# Autodesk Inventor assembly: Chasis inferior _1_
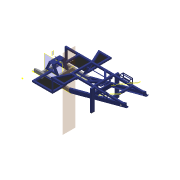
[picture p0: Inventor's stored thumbnail of the model, 180x180]
Saved by Autodesk Inventor 2020 (Build 240168000, 168)
## iProperties
Created: 2020-02-06
Part Number: Chasis inferior _1_
Document SubType Name: Assembly
Designer: Juan Carlos Botero
Author: Juan Carlos Botero
## Documents named in this file (46)
- D:\Drives\OneDrive\Carlos_2\02 TRABAJOS\MULTIPLO\Conveyor\ENSAMBLE\Chasis inferior _1_.iam
- D:\Drives\OneDrive\Carlos_2\02 TRABAJOS\MULTIPLO\Conveyor\ENSAMBLE\Refuerzo diagonal tiro.ipt
- D:\Drives\OneDrive\Carlos_2\02 TRABAJOS\MULTIPLO\Conveyor\ENSAMBLE\Lamina escalon 2.ipt
- D:\Drives\OneDrive\Carlos_2\02 TRABAJOS\MULTIPLO\Conveyor\ENSAMBLE\Lamina sujeción bateria 2.ipt
- D:\Drives\OneDrive\Carlos_2\02 TRABAJOS\MULTIPLO\Conveyor\ENSAMBLE\Refuerzo perfil en C.ipt
- D:\Drives\OneDrive\Carlos_2\02 TRABAJOS\MULTIPLO\Conveyor\ENSAMBLE\Tapa perfil 100x50.ipt
- D:\Drives\OneDrive\Carlos_2\02 TRABAJOS\MULTIPLO\Conveyor\ENSAMBLE\Angulo soporte batería 1.ipt
- D:\Drives\OneDrive\Carlos_2\02 TRABAJOS\MULTIPLO\Conveyor\ENSAMBLE\Perfil 1 en C derecho 2.ipt
- D:\Drives\OneDrive\Carlos_2\02 TRABAJOS\MULTIPLO\Conveyor\ENSAMBLE\Caucho tope banda.ipt
- D:\Drives\OneDrive\Carlos_2\02 TRABAJOS\MULTIPLO\Conveyor\ENSAMBLE\Refuerzo diagonal chasis inferior.ipt
- D:\Drives\OneDrive\Carlos_2\02 TRABAJOS\MULTIPLO\Conveyor\ENSAMBLE\Perfil escalón 6.ipt
- D:\Drives\OneDrive\Carlos_2\02 TRABAJOS\MULTIPLO\Conveyor\ENSAMBLE\Perfil escalón 3.ipt
- D:\Drives\OneDrive\Carlos_2\02 TRABAJOS\MULTIPLO\Conveyor\ENSAMBLE\Espaciador de nylon.ipt
- D:\Drives\OneDrive\Carlos_2\02 TRABAJOS\MULTIPLO\Conveyor\ENSAMBLE\Refuerzo chasis.ipt
- D:\Drives\OneDrive\Carlos_2\02 TRABAJOS\MULTIPLO\Conveyor\ENSAMBLE\Perfil escalón 4.ipt
- D:\Drives\OneDrive\Carlos_2\02 TRABAJOS\MULTIPLO\Conveyor\ENSAMBLE\Tope banda.ipt
- D:\Drives\OneDrive\Carlos_2\02 TRABAJOS\MULTIPLO\Conveyor\ENSAMBLE\Buje.ipt
- D:\Drives\OneDrive\Carlos_2\02 TRABAJOS\MULTIPLO\Conveyor\ENSAMBLE\Lamina indexacion eje trasero.ipt
- D:\Drives\OneDrive\Carlos_2\02 TRABAJOS\MULTIPLO\Conveyor\ENSAMBLE\Refuerzo horizontal tiro.ipt
- D:\Drives\OneDrive\Carlos_2\02 TRABAJOS\MULTIPLO\Conveyor\ENSAMBLE\Angulo escalón 1.ipt
- D:\Drives\OneDrive\Carlos_2\02 TRABAJOS\MULTIPLO\Conveyor\ENSAMBLE\Base chasis inferior izquierdo.ipt
- D:\Drives\OneDrive\Carlos_2\02 TRABAJOS\MULTIPLO\Conveyor\ENSAMBLE\Refuerzo diagonal estructura tiro.ipt
- D:\Drives\OneDrive\Carlos_2\02 TRABAJOS\MULTIPLO\Conveyor\ENSAMBLE\Perfil 1 en C izquierdo 2.ipt
- D:\Drives\OneDrive\Carlos_2\02 TRABAJOS\MULTIPLO\Conveyor\ENSAMBLE\Lamina escalon 1.ipt
- D:\Drives\OneDrive\Carlos_2\02 TRABAJOS\MULTIPLO\Conveyor\ENSAMBLE\Lamina pivote actuador lineal pequeño.ipt
- D:\Drives\OneDrive\Carlos_2\02 TRABAJOS\MULTIPLO\Conveyor\ENSAMBLE\Perfil 1 en C izquierdo 1.ipt
- D:\Drives\OneDrive\Carlos_2\02 TRABAJOS\MULTIPLO\Conveyor\ENSAMBLE\Perfil 1 en C derecho 1.ipt
- D:\Drives\OneDrive\Carlos_2\02 TRABAJOS\MULTIPLO\Conveyor\ENSAMBLE\Perfil escalón 2.ipt
- D:\Drives\OneDrive\Carlos_2\02 TRABAJOS\MULTIPLO\Conveyor\ENSAMBLE\Espaciador pivote 1.ipt
- D:\Drives\OneDrive\Carlos_2\02 TRABAJOS\MULTIPLO\Conveyor\ENSAMBLE\Platina inferior actuador lineal.ipt
- D:\Drives\OneDrive\Carlos_2\02 TRABAJOS\MULTIPLO\Conveyor\ENSAMBLE\Angulo escalón 3.ipt
- D:\Drives\OneDrive\Carlos_2\02 TRABAJOS\MULTIPLO\Conveyor\ENSAMBLE\Refuerzo diagonal.ipt
- D:\Drives\OneDrive\Carlos_2\02 TRABAJOS\MULTIPLO\Conveyor\ENSAMBLE\Perfil escalón 1.ipt
- D:\Drives\OneDrive\Carlos_2\02 TRABAJOS\MULTIPLO\Conveyor\ENSAMBLE\Pie amigo lamina quinta rueda.ipt
- D:\Drives\OneDrive\Carlos_2\02 TRABAJOS\MULTIPLO\Conveyor\ENSAMBLE\Lamina pivote quinta rueda.ipt
- D:\Drives\OneDrive\Carlos_2\02 TRABAJOS\MULTIPLO\Conveyor\ENSAMBLE\Angulo soporte batería 3.ipt
- D:\Drives\OneDrive\Carlos_2\02 TRABAJOS\MULTIPLO\Conveyor\ENSAMBLE\Angulo soporte batería 2.ipt
- D:\Drives\OneDrive\Carlos_2\02 TRABAJOS\MULTIPLO\Conveyor\ENSAMBLE\Unión base chasis inferior.ipt
- D:\Drives\OneDrive\Carlos_2\02 TRABAJOS\MULTIPLO\Conveyor\ENSAMBLE\Base chasis inferior derecho.ipt
- D:\Drives\OneDrive\Carlos_2\02 TRABAJOS\MULTIPLO\Conveyor\ENSAMBLE\Refuerzo intermedio.ipt
- D:\Drives\OneDrive\Carlos_2\02 TRABAJOS\MULTIPLO\Conveyor\ENSAMBLE\Ensamble cuñas y soporte _1_.iam
- D:\Drives\OneDrive\Carlos_2\02 TRABAJOS\MULTIPLO\Conveyor\ENSAMBLE\Ensamble cuñas y soporte _1__1.iam
- D:\Drives\OneDrive\Carlos_2\02 TRABAJOS\MULTIPLO\Conveyor\ENSAMBLE\sketch.ipt
- D:\Drives\OneDrive\Carlos_2\02 TRABAJOS\MULTIPLO\Conveyor\ENSAMBLE\Perfil 1 en C derecho 2_MIR.ipt
- D:\Drives\OneDrive\Carlos_2\02 TRABAJOS\MULTIPLO\Paral_baliza.iam
- D:\Drives\OneDrive\Carlos_2\02 TRABAJOS\MULTIPLO\Conveyor\ENSAMBLE - Copy\Modificacion_altura.iam
## Components (80 placed, 44 different names)
1. Refuerzo diagonal tiro:1
2. Lamina escalon 2:1
3. Lamina sujeción bateria 2:1
4. Lamina escalon 2:2
5. Refuerzo perfil en C:1
6. Tapa perfil 100x50:1
7. Angulo soporte batería 1:1
8. Perfil 1 en C derecho 2:1
9. Caucho tope banda:1
10. Refuerzo diagonal chasis inferior:1
11. Perfil escalón 6:1
12. Refuerzo perfil en C:2
13. Espaciador de nylon:1
14. Perfil escalón 4:1
15. Tope banda:1
16. Buje:1
17. Perfil escalón 3:2
18. Lamina indexacion eje trasero:1
19. Refuerzo horizontal tiro:1
20. Angulo escalón 1:1
21. Base chasis inferior izquierdo:1
22. Perfil escalón 3:3
23. Lamina indexacion eje trasero:2
24. Refuerzo horizontal tiro:2 — Flush:7
25. Caucho tope banda:2
26. Refuerzo diagonal estructura tiro:1
27. Refuerzo diagonal tiro:2
28. Perfil 1 en C izquierdo 2:1
29. Tapa perfil 100x50:2
30. Refuerzo diagonal chasis inferior:2
31. Lamina escalon 1:1
32. Lamina pivote actuador lineal pequeño:1
33. Perfil 1 en C izquierdo 1:1
34. Perfil 1 en C derecho 1:1
35. Perfil escalón 2:1 — Flush:14, Flush:15
36. Lamina pivote actuador lineal pequeño:2
37. Espaciador pivote 1:1
38. Refuerzo chasis:2
39. Perfil escalón 3:4
40. Platina inferior actuador lineal:1
41. Espaciador pivote 1:2
42. Buje:3
43. Perfil escalón 3:5
44. Angulo escalón 3:1
45. Refuerzo diagonal:1
46. Espaciador de nylon:3
47. Refuerzo diagonal estructura tiro:2 — Flush:7
48. Perfil escalón 1:1
49. Pie amigo lamina quinta rueda:1
50. Tapa perfil 100x50:3
51. Perfil escalón 4:2
52. Refuerzo diagonal:2
53. Angulo escalón 3:2
54. Pie amigo lamina quinta rueda:2
55. Platina inferior actuador lineal:2
56. Tope banda:2
57. Tapa perfil 100x50:4
58. Platina inferior actuador lineal:3
59. Pie amigo lamina quinta rueda:3
60. Lamina pivote quinta rueda:1
61. Angulo soporte batería 3:1
62. Angulo soporte batería 2:1
63. Perfil escalón 2:2
64. Angulo soporte batería 3:2
65. Pie amigo lamina quinta rueda:4
66. Unión base chasis inferior:1
67. Perfil escalón 6:2
68. Lamina escalon 1:2
69. Base chasis inferior derecho:1
70. Angulo escalón 1:2
71. Refuerzo intermedio:1
72. Perfil escalón 1:2 — Mate:9
73. Refuerzo intermedio:2
74. Platina inferior actuador lineal:4
75. Ensamble cuñas y soporte <1>:1 [sub-assembly]
76. Ensamble cuñas y soporte <1>:2 [sub-assembly]
77. sketch:1 — Flush:1
78. Perfil 1 en C derecho 2_MIR:1
79. Paral_baliza:1 [sub-assembly] — Mate:9, Flush:14, Flush:15
80. Modificacion_altura:1 [sub-assembly]
## Relationships (12: Flush 6, Mate 6)
- Flush:1: sketch:1
- Flush:7: Refuerzo horizontal tiro:2 ↔ Refuerzo diagonal estructura tiro:2
- Mate:9: Perfil escalón 1:2 ↔ Paral_baliza:1
- Flush:14: Perfil escalón 2:1 ↔ Paral_baliza:1
- Flush:15: Perfil escalón 2:1 ↔ Paral_baliza:1
- [Flush]: Modificacion_altura:1
- [Mate]: Perfil escalón 1:1 ↔ Modificacion_altura:1
- [Flush] (-25 mm): Perfil 1 en C derecho 2_MIR:1 ↔ Modificacion_altura:1
- [Mate]: Perfil 1 en C izquierdo 2:1 ↔ Modificacion_altura:1
- [Mate]: Modificacion_altura:1
- [Mate]: Refuerzo diagonal estructura tiro:1 ↔ Modificacion_altura:1
- [Mate]: Refuerzo diagonal estructura tiro:1 ↔ Modificacion_altura:1
